# Autodesk Inventor assembly: Assembly Mast
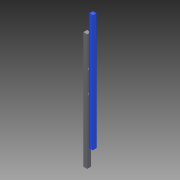
[picture p0: Inventor's stored thumbnail of the model, 180x180]
Saved by Autodesk Inventor 2015 (Build 190159000, 159)
## iProperties
Created: 2016-01-11
Part Number: Assembly Mast
Document SubType Name: Assembly
Designer: Applegate
Author: Applegate
## Documents named in this file (3)
- C:\Users\Applegate\Desktop\Chassy Files\Mast\Assembly Mast.iam
- C:\Users\Applegate\Desktop\Chassy Files\Mast\Main.ipt
- C:\Users\Applegate\Desktop\Chassy Files\Mast\gear.ipt
## Components (4 placed, 2 different names)
1. Main:1 — Tangent:1, Tangent:2, Flush:1, Flush:2, Rotation/Translation:3, Rotation/Translation:4
2. gear:4 — Tangent:1, Flush:2, Tangent:4, Rotation/Translation:2, Rotation/Translation:4
3. gear:5 — Tangent:2, Flush:1, Tangent:3, Flush:3, Rotation/Translation:1, Rotation/Translation:3
4. Main:2 — Tangent:3, Flush:3, Tangent:4, Rotation/Translation:1, Rotation/Translation:2
## Relationships (11: Tangent 4, RelateRotateTranslate 4, Flush 3)
- Tangent:1: Main:1 ↔ gear:4
- Tangent:2: Main:1 ↔ gear:5
- Flush:1: Main:1 ↔ gear:5
- Flush:2: Main:1 ↔ gear:4
- Tangent:3: gear:5 ↔ Main:2
- Flush:3: gear:5 ↔ Main:2
- Tangent:4: gear:4 ↔ Main:2
- Rotation/Translation:1 [RelateRotateTranslate] (25.4 mm): gear:5 ↔ Main:2
- Rotation/Translation:2 [RelateRotateTranslate] (25.4 mm): gear:4 ↔ Main:2
- Rotation/Translation:3 [RelateRotateTranslate] (25.4 mm): Main:1 ↔ gear:5
- Rotation/Translation:4 [RelateRotateTranslate] (25.4 mm): Main:1 ↔ gear:4
